# Autodesk Inventor assembly: Bin Options
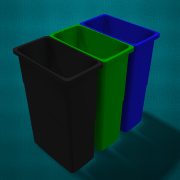
[picture p0: Inventor's stored thumbnail of the model, 180x180]
Saved by Autodesk Inventor 2017 (Build 210142000, 142)
## iProperties
Created: 2017-10-01
Part Number: Bin Options
Document SubType Name: Assembly
Designer: MMoreno
Author: MMoreno
## Documents named in this file (4)
- C:\Users\Michael\Google Drive\Businesses\Xatie Corp\Porfolio Pieces\Trash Can\Bin Options.iam
- C:\Users\Michael\Google Drive\Businesses\Xatie Corp\Porfolio Pieces\Trash Can\Recycle Bin.ipt
- C:\Users\Michael\Google Drive\Businesses\Xatie Corp\Porfolio Pieces\Trash Can\Waste Bin.ipt
- C:\Users\Michael\Google Drive\Businesses\Xatie Corp\Porfolio Pieces\Trash Can\Organic Bin.ipt
## Components (3 placed, 3 different names)
1. Recycle Bin:1 — Flush:2, Flush:3, Mate:2
2. Waste Bin:1 — Flush:1, Flush:2, Flush:3, Flush:4, Mate:1
3. Organic Bin:1 — Flush:1, Flush:4, Mate:1, Mate:2
## Relationships (6: Flush 4, Mate 2)
- Flush:1: Waste Bin:1 ↔ Organic Bin:1
- Flush:2: Recycle Bin:1 ↔ Waste Bin:1
- Flush:3: Recycle Bin:1 ↔ Waste Bin:1
- Flush:4: Waste Bin:1 ↔ Organic Bin:1
- Mate:1: Waste Bin:1 ↔ Organic Bin:1
- Mate:2: Recycle Bin:1 ↔ Organic Bin:1
